# Autodesk Inventor assembly: SUBDriveShaftACME
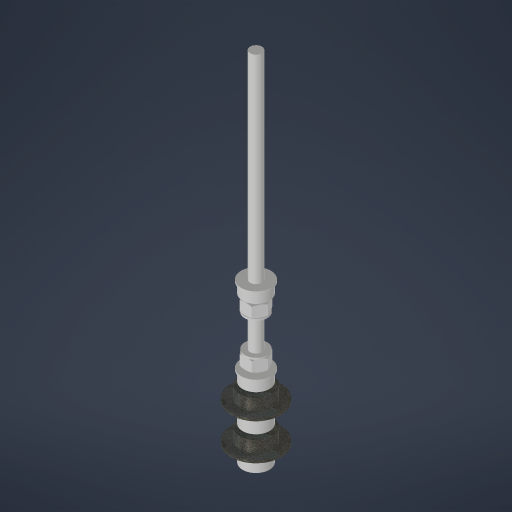
[picture p0: Inventor's stored thumbnail of the model, 512x512]
Saved by Autodesk Inventor 2024 (Build 280153000, 153)
## iProperties
Created: 2025-02-08
Part Number: SUBDriveShaftACME
Document SubType Name: Assembly
Designer: Tommy Rohmann
Author: Tommy Rohmann
## Documents named in this file (9)
- C:\Users\Tommy Rohmann\OneDrive\Projects\Microgravity-Press-Washing-Machine\System Design and Documentation\Inventor Design Project\SUBDriveShaftACME.iam
- C:\Users\Tommy Rohmann\OneDrive\Projects\Microgravity-Press-Washing-Machine\System Design and Documentation\Inventor Design Project\LoadCell.ipt
- C:\Users\Tommy Rohmann\OneDrive\Projects\Microgravity-Press-Washing-Machine\System Design and Documentation\Inventor Design Project\ACMEHexNut.ipt
- C:\Users\Tommy Rohmann\OneDrive\Projects\Microgravity-Press-Washing-Machine\System Design and Documentation\Inventor Design Project\DriveSprocket.ipt
- C:\Users\Tommy Rohmann\OneDrive\Projects\Microgravity-Press-Washing-Machine\System Design and Documentation\Inventor Design Project\FlangedJournalBearing.ipt
- C:\Users\Tommy Rohmann\OneDrive\Projects\Microgravity-Press-Washing-Machine\System Design and Documentation\Inventor Design Project\ScrewDriveSprocket.ipt
- C:\Users\Tommy Rohmann\OneDrive\Projects\Microgravity-Press-Washing-Machine\System Design and Documentation\Inventor Design Project\ThrustBearing.ipt
- C:\Users\Tommy Rohmann\OneDrive\Projects\Microgravity-Press-Washing-Machine\System Design and Documentation\Inventor Design Project\ACMEScrew.ipt
- C:\Users\Tommy Rohmann\OneDrive\Projects\Microgravity-Press-Washing-Machine\System Design and Documentation\Inventor Design Project\TensionerSprocket.ipt
## Components (15 placed, 8 different names)
1. LoadCell:1 — Mate:27, Mate:28, Mate:29
2. ACMEHexNut:1 — Mate:8, Mate:11, Mate:12
3. DriveSprocket:1 — Flush:1
4. FlangedJournalBearing:1 — Mate:9, Mate:10, Mate:30
5. ScrewDriveSprocket:1 — Mate:13, Mate:14, Flush:1, Mate:16, Flush:5
6. ThrustBearing:1 — Mate:8, Mate:25, Mate:28
7. ThrustBearing:2 — Mate:6, Mate:26, Mate:27
8. ACMEHexNut:2 — Mate:6, Mate:9, Mate:10
9. FlangedJournalBearing:2 — Mate:11, Mate:12, Mate:13, Mate:14, Mate:31
10. FlangedJournalBearing:3 — Mate:16, Mate:18, Mate:20, Mate:23
11. ScrewDriveSprocket:2 — Mate:18, Mate:20, Flush:6
12. FlangedJournalBearing:4 — Flush:4, Mate:24
13. ACMEScrew:1 — Flush:4, Mate:25, Mate:26, Mate:29, Mate:30, Mate:31
14. TensionerSprocket:1 — Flush:5, Mate:23
15. TensionerSprocket:2 — Flush:6, Mate:24
## Relationships (25: Mate 21, Flush 4)
- Mate:6: ThrustBearing:2 ↔ ACMEHexNut:2
- Mate:8: ACMEHexNut:1 ↔ ThrustBearing:1
- Mate:9 (3.175 mm): FlangedJournalBearing:1 ↔ ACMEHexNut:2
- Mate:10: FlangedJournalBearing:1 ↔ ACMEHexNut:2
- Mate:11 (3.175 mm): ACMEHexNut:1 ↔ FlangedJournalBearing:2
- Mate:12: ACMEHexNut:1 ↔ FlangedJournalBearing:2
- Mate:13 (3.175 mm): ScrewDriveSprocket:1 ↔ FlangedJournalBearing:2
- Mate:14: ScrewDriveSprocket:1 ↔ FlangedJournalBearing:2
- Flush:1: DriveSprocket:1 ↔ ScrewDriveSprocket:1
- Mate:16: ScrewDriveSprocket:1 ↔ FlangedJournalBearing:3
- [Mate]: ScrewDriveSprocket:2 ↔ FlangedJournalBearing:4
- Mate:18: FlangedJournalBearing:3 ↔ ScrewDriveSprocket:2
- Mate:20 (3.175 mm): FlangedJournalBearing:3 ↔ ScrewDriveSprocket:2
- Flush:4: FlangedJournalBearing:4 ↔ ACMEScrew:1
- Flush:5: ScrewDriveSprocket:1 ↔ TensionerSprocket:1
- Mate:23 (3.175 mm): FlangedJournalBearing:3 ↔ TensionerSprocket:1
- Flush:6: ScrewDriveSprocket:2 ↔ TensionerSprocket:2
- Mate:24: FlangedJournalBearing:4 ↔ TensionerSprocket:2
- Mate:25: ThrustBearing:1 ↔ ACMEScrew:1
- Mate:26: ThrustBearing:2 ↔ ACMEScrew:1
- Mate:27: LoadCell:1 ↔ ThrustBearing:2
- Mate:28: LoadCell:1 ↔ ThrustBearing:1
- Mate:29: LoadCell:1 ↔ ACMEScrew:1
- Mate:30: FlangedJournalBearing:1 ↔ ACMEScrew:1
- Mate:31: FlangedJournalBearing:2 ↔ ACMEScrew:1
## Named parameters: d18_d17 = 0 mm
